# Autodesk Inventor assembly: Helix DLP V2
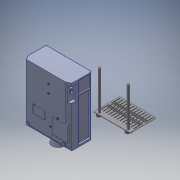
[picture p0: Inventor's stored thumbnail of the model, 180x180]
Saved by Autodesk Inventor 2019 (Build 230136000, 136)
## iProperties
Created: 2020-11-30
Part Number: Helix DLP V2
Document SubType Name: Assembly
Designer: Vijay
Author: Vijay
## Documents named in this file (5)
- C:\Users\Vijay\Documents\GitHub\Helix-DLP-3D-Printer\Helix DLP V2\Helix DLP V2.iam
- C:\Users\Vijay\Documents\GitHub\Helix-DLP-3D-Printer\Helix DLP V2\OTS Componenets\Projector.ipt
- C:\Users\Vijay\Documents\GitHub\Helix-DLP-3D-Printer\Helix DLP V2\Build Plate.ipt
- C:\Users\Vijay\Documents\GitHub\Helix-DLP-3D-Printer\Helix DLP V2\Z Shaft.ipt
- C:\Users\Vijay\Documents\GitHub\Helix-DLP-3D-Printer\Helix DLP V2\OTS Componenets\108110252-9-support_shf16\support_shf16.ipt
## Components (6 placed, 4 different names)
1. Projector:1
2. Build Plate:1 — Mate:3, Flush:4, Flush:5
3. Z Shaft:1 — Mate:1, Flush:1
4. Z Shaft:2 — Mate:2, Flush:2
5. support_shf16:1 — Mate:1, Flush:1, Flush:3, Mate:3, Flush:4
6. support_shf16:2 — Mate:2, Flush:2, Flush:3, Flush:5
## Relationships (8: Flush 5, Mate 3)
- Mate:1: Z Shaft:1 ↔ support_shf16:1
- Mate:2: Z Shaft:2 ↔ support_shf16:2
- Flush:1: Z Shaft:1 ↔ support_shf16:1
- Flush:2: Z Shaft:2 ↔ support_shf16:2
- Flush:3: support_shf16:1 ↔ support_shf16:2
- Mate:3: Build Plate:1 ↔ support_shf16:1
- Flush:4: Build Plate:1 ↔ support_shf16:1
- Flush:5: Build Plate:1 ↔ support_shf16:2
